# Autodesk Inventor assembly: PitchAssembly
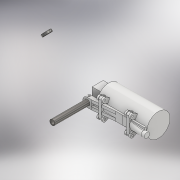
[picture p0: Inventor's stored thumbnail of the model, 180x180]
Saved by Autodesk Inventor 2018 (Build 220112000, 112)
## iProperties
Created: 2018-03-26
Part Number: PitchAssembly
Document SubType Name: Assembly
Designer: mansu
Author: mansu
## Documents named in this file (5)
- F:\OneDrive\Documents\2018 UBC\ELEC 391\Controller\cad\release\PitchAssemblyC.iam
- F:\OneDrive\Documents\2018 UBC\ELEC 391\Controller\cad\release\Rod3_8in.ipt
- F:\OneDrive\Documents\2018 UBC\ELEC 391\Controller\cad\release\R1038_ZZ_W Bearing.ipt
- F:\OneDrive\Documents\2018 UBC\ELEC 391\Controller\cad\release\PitchMotor\MockPitchMotor.ipt
- F:\OneDrive\Documents\2018 UBC\ELEC 391\Controller\cad\release\ShaftArmC.ipt
## Components (4 placed, 4 different names)
1. Rod3_8in:1 — Mate:9, Mate:10
2. R1038_ZZ_W Bearing:1
3. MockPitchMotor:1 — Mate:11, Mate:12, Mate:13
4. ShaftArmC:1 — Mate:10, Mate:11, Mate:12, Mate:13
## Relationships (5: Mate 5)
- Mate:9: Rod3_8in:1
- Mate:10: Rod3_8in:1 ↔ ShaftArmC:1
- Mate:11: MockPitchMotor:1 ↔ ShaftArmC:1
- Mate:12: MockPitchMotor:1 ↔ ShaftArmC:1
- Mate:13: MockPitchMotor:1 ↔ ShaftArmC:1
